# Autodesk Inventor assembly: +XPanel
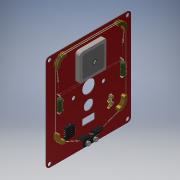
[picture p0: Inventor's stored thumbnail of the model, 180x180]
Saved by Autodesk Inventor 2018 (Build 220112000, 112)
## iProperties
Created: 2018-10-25
Part Number: +XPanel
Document SubType Name: Assembly
Designer: Bradley
Author: Bradley
## Documents named in this file (16)
- C:\Users\Bradley\Documents\GitHub\CougSat1-Hardware\CougSat1-RadioBoard\CADModel\Native\+XPanel.iam
- C:\Users\Bradley\Documents\GitHub\CougSat1-Hardware\CougSat1-RadioBoard\CADModel\Native\+XPanel_PCB.ipt
- C:\Users\Bradley\Documents\GitHub\Resources\ComponentModels\Electronics\Antenna_GPSPatch.ipt
- C:\Users\Bradley\Documents\GitHub\Resources\ComponentModels\Connectors\U.FL_Male.ipt
- C:\Users\Bradley\Documents\GitHub\Resources\ComponentModels\Electronics\Resistor_TH-15mm.ipt
- C:\Users\Bradley\Documents\GitHub\CougSat1-Hardware\CougSat1-RadioBoard\CADModel\Native\+XPanel_AntennaPost.ipt
- C:\Users\Bradley\Documents\GitHub\Resources\ComponentModels\Fasteners\Bolt_M2x0.4_4mm_SH.ipt
- C:\Users\Bradley\Documents\GitHub\Resources\ComponentModels\Fasteners\Nut_SMD_M2x0.4_1mm.ipt
- C:\Users\Bradley\Documents\GitHub\CougSat1-Hardware\CougSat1-RadioBoard\CADModel\Native\+XPanel_AntennaMount.ipt
- C:\Users\Bradley\Documents\GitHub\Resources\ComponentModels\Connectors\PicoLock-J-4.ipt
- C:\Users\Bradley\Documents\GitHub\Resources\ComponentModels\Connectors\PicoLock-P-4.ipt
- C:\Users\Bradley\Documents\GitHub\Resources\ComponentModels\Connectors\U.FL_Female.ipt
- C:\Users\Bradley\Documents\GitHub\CougSat1-Hardware\CougSat1-RadioBoard\CADModel\Native\+XPanel_AntennaStored+Y.ipt
- C:\Users\Bradley\Documents\GitHub\CougSat1-Hardware\CougSat1-RadioBoard\CADModel\Native\+XPanel_AntennaStored-Y.ipt
- C:\Users\Bradley\Documents\GitHub\CougSat1-Hardware\CougSat1-RadioBoard\CADModel\Native\+XPanel_AntennaString.ipt
- C:\Users\Bradley\Documents\GitHub\CougsInSpace\CougSat1-Hardware\CougSat1-RadioBoard\CADModel\Native\+XPanel_AntennaDeployed.ipt
## Components (25 placed, 15 different names)
1. +XPanel_AntennaDeployed:1 — Mate:24, Mate:25
2. +XPanel_AntennaDeployed:2 — Mate:26, Mate:27
3. +XPanel_AntennaMount:1 — Insert:11, Insert:12, Insert:13, Insert:14, Mate:25, Mate:27
4. +XPanel_AntennaPost:1 — Insert:4, Mate:9
5. +XPanel_AntennaPost:2 — Insert:8, Mate:10
6. +XPanel_AntennaPost:3 — Insert:7, Mate:11, Mate:13, Mate:17
7. +XPanel_AntennaPost:4 — Insert:6, Mate:12, Mate:15, Mate:16
8. +XPanel_AntennaStored+Y:1 — Mate:13, Mate:14, Mate:15
9. +XPanel_AntennaStored-Y:1 — Mate:16, Mate:17, Mate:18
10. +XPanel_AntennaString:1 — Mate:19, Mate:20, Flush:6
11. +XPanel_AntennaString:2 — Mate:21, Mate:22, Mate:23
12. +XPanel_PCB:1 — Insert:1, Mate:1, Mate:2, Insert:4, Insert:6, Insert:7, Insert:8, Insert:9, Insert:10, Insert:11, Insert:12, Mate:5, Mate:9, Mate:10, Mate:11, Mate:12, Mate:14, Mate:18, Insert:17, Insert:18, Insert:19, Insert:20, Mate:24, Mate:26
13. PicoLock-J-4:1 — Mate:5, Flush:3, Mate:6
14. PicoLock-P-4:1
15. U.FL_Female:1 — Insert:16, Angle:1
16. U.FL_Female:2 — Insert:15, Angle:2
17. U.FL_Male:1 — Mate:1, Mate:7, Flush:4, Insert:16
18. U.FL_Male:2 — Mate:2, Flush:5, Mate:8, Insert:15
19. Antenna_GPSPatch:1 — Insert:1, Flush:1
20. Resistor_TH-15mm:1 — Insert:17, Insert:18, Mate:19, Mate:23
21. Resistor_TH-15mm:2 — Insert:19, Insert:20, Mate:20, Mate:22
22. Bolt_M2x0.4_4mm_SH:1 — Insert:13
23. Bolt_M2x0.4_4mm_SH:2 — Insert:14
24. Nut_SMD_M2x0.4_1mm:1 — Insert:9
25. Nut_SMD_M2x0.4_1mm:2 — Insert:10
## Relationships (52: Mate 27, Insert 17, Flush 6, Angle 2)
- Insert:1: +XPanel_PCB:1 ↔ Antenna_GPSPatch:1
- Flush:1: Antenna_GPSPatch:1
- Mate:1: +XPanel_PCB:1 ↔ U.FL_Male:1
- Mate:2: +XPanel_PCB:1 ↔ U.FL_Male:2
- Insert:4: +XPanel_AntennaPost:1 ↔ +XPanel_PCB:1
- Insert:6: +XPanel_AntennaPost:4 ↔ +XPanel_PCB:1
- Insert:7: +XPanel_AntennaPost:3 ↔ +XPanel_PCB:1
- Insert:8: +XPanel_AntennaPost:2 ↔ +XPanel_PCB:1
- Insert:9: +XPanel_PCB:1 ↔ Nut_SMD_M2x0.4_1mm:1
- Insert:10: +XPanel_PCB:1 ↔ Nut_SMD_M2x0.4_1mm:2
- Insert:11: +XPanel_AntennaMount:1 ↔ +XPanel_PCB:1
- Insert:12: +XPanel_AntennaMount:1 ↔ +XPanel_PCB:1
- Insert:13: +XPanel_AntennaMount:1 ↔ Bolt_M2x0.4_4mm_SH:1
- Insert:14: +XPanel_AntennaMount:1 ↔ Bolt_M2x0.4_4mm_SH:2
- [Flush]: PicoLock-J-4:1 ↔ PicoLock-P-4:1
- [Mate]: PicoLock-J-4:1 ↔ PicoLock-P-4:1
- [Mate] (0.025 mm): PicoLock-J-4:1 ↔ PicoLock-P-4:1
- Mate:5: +XPanel_PCB:1 ↔ PicoLock-J-4:1
- Flush:3 (23 mm): PicoLock-J-4:1
- Mate:6 (-24 mm): PicoLock-J-4:1
- Mate:7 (20 mm): U.FL_Male:1
- Flush:4 (20 mm): U.FL_Male:1
- Flush:5 (15 mm): U.FL_Male:2
- Mate:8 (20 mm): U.FL_Male:2
- Insert:15 (0.1 mm): U.FL_Female:2 ↔ U.FL_Male:2
- Insert:16 (0.1 mm): U.FL_Female:1 ↔ U.FL_Male:1
- Angle:1 (30 deg): U.FL_Female:1
- Angle:2 (30 deg): U.FL_Female:2
- Mate:9: +XPanel_AntennaPost:1 ↔ +XPanel_PCB:1
- Mate:10: +XPanel_AntennaPost:2 ↔ +XPanel_PCB:1
- Mate:11: +XPanel_AntennaPost:3 ↔ +XPanel_PCB:1
- Mate:12: +XPanel_AntennaPost:4 ↔ +XPanel_PCB:1
- Mate:13: +XPanel_AntennaPost:3 ↔ +XPanel_AntennaStored+Y:1
- Mate:14 (2.5 mm): +XPanel_AntennaStored+Y:1 ↔ +XPanel_PCB:1
- Mate:15: +XPanel_AntennaPost:4 ↔ +XPanel_AntennaStored+Y:1
- Mate:16: +XPanel_AntennaPost:4 ↔ +XPanel_AntennaStored-Y:1
- Mate:17: +XPanel_AntennaPost:3 ↔ +XPanel_AntennaStored-Y:1
- Mate:18 (1 mm): +XPanel_AntennaStored-Y:1 ↔ +XPanel_PCB:1
- Insert:17 (-1 mm): +XPanel_PCB:1 ↔ Resistor_TH-15mm:1
- Insert:18 (-1 mm): +XPanel_PCB:1 ↔ Resistor_TH-15mm:1
- Insert:19 (-1 mm): +XPanel_PCB:1 ↔ Resistor_TH-15mm:2
- Insert:20 (-1 mm): +XPanel_PCB:1 ↔ Resistor_TH-15mm:2
- Mate:19: +XPanel_AntennaString:1 ↔ Resistor_TH-15mm:1
- Mate:20: +XPanel_AntennaString:1 ↔ Resistor_TH-15mm:2
- Flush:6 (2.8 mm): +XPanel_AntennaString:1
- Mate:21 (1.3 mm): +XPanel_AntennaString:2
- Mate:22: +XPanel_AntennaString:2 ↔ Resistor_TH-15mm:2
- Mate:23: +XPanel_AntennaString:2 ↔ Resistor_TH-15mm:1
- Mate:24: +XPanel_AntennaDeployed:1 ↔ +XPanel_PCB:1
- Mate:25: +XPanel_AntennaDeployed:1 ↔ +XPanel_AntennaMount:1
- Mate:26: +XPanel_AntennaDeployed:2 ↔ +XPanel_PCB:1
- Mate:27: +XPanel_AntennaDeployed:2 ↔ +XPanel_AntennaMount:1
## Named parameters: d105_d9 = 0 mm, d106_d10 = 0 mm, d107_d11 = 0.025 mm
